# Autodesk Inventor assembly: ㄷ자 프레임 샘플
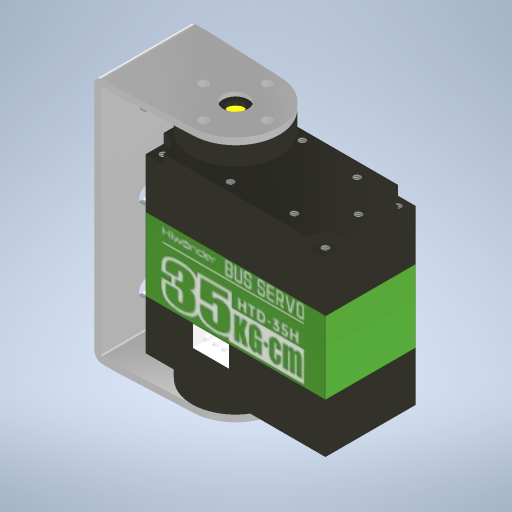
[picture p0: Inventor's stored thumbnail of the model, 512x512]
Saved by Autodesk Inventor 2023 (Build 270158000, 158)
## iProperties
Created: 2022-10-22
Part Number: ㄷ자 프레임 샘플
Document SubType Name: Assembly
Designer: chanh
Author: chanh
## Documents named in this file (5)
- C:\Users\chanh\OneDrive - 연세대학교 (Yonsei University)\로봇\Humanoid\Roboin Humanoid Project\Inventor\2-Axis Manipulator\Designs\Assembly\ㄷ자 프레임 샘플.iam
- C:\Users\chanh\OneDrive - 연세대학교 (Yonsei University)\로봇\Humanoid\Roboin Humanoid Project\Inventor\2-Axis Manipulator\Designs\Part\servo.ipt
- C:\Users\chanh\OneDrive - 연세대학교 (Yonsei University)\로봇\Humanoid\Roboin Humanoid Project\Inventor\2-Axis Manipulator\Designs\Part\servo-horn_bottom.ipt
- C:\Users\chanh\OneDrive - 연세대학교 (Yonsei University)\로봇\Humanoid\Roboin Humanoid Project\Inventor\2-Axis Manipulator\Designs\Part\servo-horn_top.ipt
- C:\Users\chanh\OneDrive - 연세대학교 (Yonsei University)\로봇\Humanoid\Roboin Humanoid Project\Inventor\2-Axis Manipulator\Designs\Part\ㄷ_frame_1.ipt
## Components (4 placed, 4 different names)
1. servo:1 — Flush:1, Flush:2, Flush:3, Rotational:1
2. servo-horn_bottom:1 — Rigid:1
3. servo-horn_top:1 — Rotational:1, Rigid:2
4. ㄷ_frame_1:1 — Rigid:1, Rigid:2
## Relationships (6: Flush 3, WeldJoint 2, RevoluteJoint 1)
- Flush:1: servo:1
- Flush:2: servo:1
- Flush:3: servo:1
- Rotational:1 [RevoluteJoint] (0.9 mm): servo:1 ↔ servo-horn_top:1
- Rigid:1 [WeldJoint]: servo-horn_bottom:1 ↔ ㄷ_frame_1:1
- Rigid:2 [WeldJoint]: servo-horn_top:1 ↔ ㄷ_frame_1:1
